# Autodesk Inventor assembly: Cover-Frame-Assembly
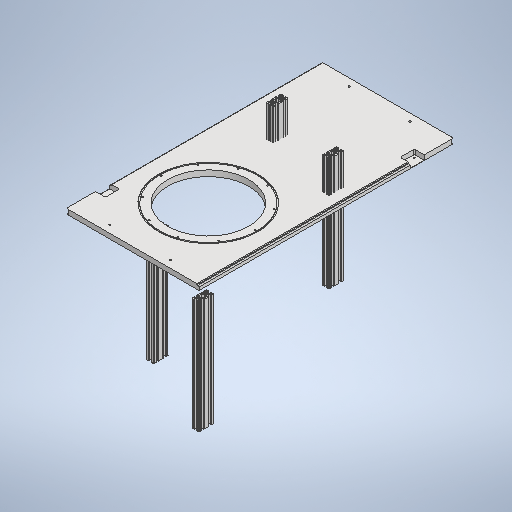
[picture p0: Inventor's stored thumbnail of the model, 512x512]
Saved by Autodesk Inventor 2025 (Build 290162000, 162)
## iProperties
Created: 2024-06-18
Part Number: Cover-Frame-Assembly
Document SubType Name: Assembly
Designer: mumin
Author: mumin
## Documents named in this file (3)
- C:\GitHub\In-situ-monitoring-of-powder-bed-fusion-additive-manufacturing\system_development\Orichalcum\v0.2\Hardware_design\custom-cover\Cover-Frame-Assembly.iam
- C:\GitHub\In-situ-monitoring-of-powder-bed-fusion-additive-manufacturing\system_development\Orichalcum\v0.2\Hardware_design\custom-cover\cover\Updated Cover.ipt
- C:\GitHub\In-situ-monitoring-of-powder-bed-fusion-additive-manufacturing\system_development\Orichalcum\v0.2\Hardware_design\custom-cover\8020-parts\20-40.ipt
## Components (5 placed, 2 different names)
1. Updated Cover:1 — Mate:1, Flush:1, Flush:2
2. 20-40:1 — Mate:1, Flush:1, Flush:2
3. 20-40:2
4. 20-40:3
5. 20-40:4
## Relationships (3: Flush 2, Mate 1)
- Mate:1: Updated Cover:1 ↔ 20-40:1
- Flush:1: Updated Cover:1 ↔ 20-40:1
- Flush:2: Updated Cover:1 ↔ 20-40:1
